# Autodesk Inventor assembly: axis_module_v2
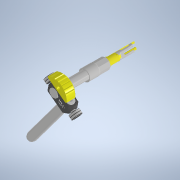
[picture p0: Inventor's stored thumbnail of the model, 180x180]
Saved by Autodesk Inventor 2022 (Build 260153000, 153)
## iProperties
Created: 2021-02-07
Part Number: axis_module_v2
Document SubType Name: Assembly
Designer: dsdan
Author: dsdan
## Documents named in this file (8)
- E:\OneDrive - Imperial College London\DragonVision_DanielKo\Instrumentation\Ephys_rig_2021\axis_module_v2.iam
- E:\OneDrive - Imperial College London\DragonVision_DanielKo\Instrumentation\Ephys_rig_2021\Imported Components\TR100_M-Solidworks.ipt
- E:\OneDrive - Imperial College London\DragonVision_DanielKo\Instrumentation\Ephys_rig_2021\tool_adapter_3.ipt
- E:\OneDrive - Imperial College London\DragonVision_DanielKo\Instrumentation\Ephys_rig_2021\Imported Components\RA90_M-Solidworks.ipt
- E:\OneDrive - Imperial College London\DragonVision_DanielKo\Instrumentation\Ephys_rig_2021\Imported Components\TR60_M-Solidworks.ipt
- E:\OneDrive - Imperial College London\DragonVision_DanielKo\Instrumentation\Ephys_rig_2021\Holder\dk_dorsal_v3.ipt
- E:\OneDrive - Imperial College London\DragonVision_DanielKo\Instrumentation\Ephys_rig_2021\Holder\body_adjustable_parametric_v3.ipt
- E:\OneDrive - Imperial College London\DragonVision_DanielKo\Instrumentation\Ephys_rig_2021\Holder\adapter.ipt
## Components (7 placed, 7 different names)
1. RA90_M-Solidworks:1 — Mate:48, Flush:50, Flush:51, Angle:1, Mate:49, Flush:52, Mate:50
2. TR100_M-Solidworks:2 — Mate:48, Flush:50
3. tool_adapter_3:1 — Flush:51, Angle:1, Mate:49, Mate:51
4. TR60_M-Solidworks:1 — Flush:52, Mate:50, Mate:51, Mate:53, Mate:54
5. dk_dorsal_v3:1 — Mate:56, Mate:57, Mate:58
6. body_adjustable_parametric_v3:1 — Angle:53, Mate:52, Mate:55, Mate:56, Mate:57, Mate:58
7. adapter:1 — Angle:53, Mate:52, Mate:53, Mate:54, Mate:55
## Relationships (16: Mate 11, Flush 3, Angle 2)
- Mate:48: RA90_M-Solidworks:1 ↔ TR100_M-Solidworks:2
- Flush:50: RA90_M-Solidworks:1 ↔ TR100_M-Solidworks:2
- Flush:51: RA90_M-Solidworks:1 ↔ tool_adapter_3:1
- Angle:1 (180 deg): RA90_M-Solidworks:1 ↔ tool_adapter_3:1
- Mate:49: RA90_M-Solidworks:1 ↔ tool_adapter_3:1
- Flush:52: RA90_M-Solidworks:1 ↔ TR60_M-Solidworks:1
- Mate:50: RA90_M-Solidworks:1 ↔ TR60_M-Solidworks:1
- Mate:51: tool_adapter_3:1 ↔ TR60_M-Solidworks:1
- Angle:53 (180 deg): body_adjustable_parametric_v3:1 ↔ adapter:1
- Mate:52: body_adjustable_parametric_v3:1 ↔ adapter:1
- Mate:53: TR60_M-Solidworks:1 ↔ adapter:1
- Mate:54: TR60_M-Solidworks:1 ↔ adapter:1
- Mate:55: body_adjustable_parametric_v3:1 ↔ adapter:1
- Mate:56: dk_dorsal_v3:1 ↔ body_adjustable_parametric_v3:1
- Mate:57: dk_dorsal_v3:1 ↔ body_adjustable_parametric_v3:1
- Mate:58: dk_dorsal_v3:1 ↔ body_adjustable_parametric_v3:1
